# Autodesk Inventor assembly: Backhoe
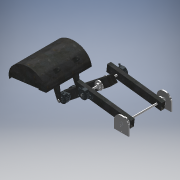
[picture p0: Inventor's stored thumbnail of the model, 180x180]
Saved by Autodesk Inventor 2019 (Build 230136000, 136)
## iProperties
Created: 2018-10-28
Part Number: Backhoe
Document SubType Name: Assembly
Designer: Alex Barnett
Author: Alex Barnett
## Documents named in this file (11)
- C:\Users\Alex Barnett\Documents\Machine Design\PR2\CAD\Backhoe.iam
- C:\Users\Alex Barnett\Documents\Machine Design\PR2\CAD\Boom Hinge.ipt
- C:\Users\Alex Barnett\Documents\Machine Design\PR2\CAD\Pin .5in. Dia. - Boom Hinge.ipt
- C:\Users\Alex Barnett\Documents\Machine Design\PR2\CAD\Ball Bearing .5in..ipt
- C:\Users\Alex Barnett\Documents\Machine Design\PR2\CAD\Steel 4130 1x2in. Tubing, t=.065in.,L=15in..ipt
- C:\Users\Alex Barnett\Documents\Machine Design\PR2\CAD\Flange-Mount Shaft Collar 0.5in..ipt
- C:\Users\Alex Barnett\Documents\Machine Design\PR2\CAD\Steel 4130 1x2in. Tubing, t=.065in.,L=22in..ipt
- C:\Users\Alex Barnett\Documents\Machine Design\PR2\CAD\Flange-Mount Sealed Ball Bearing .5in. Dia..ipt
- C:\Users\Alex Barnett\Documents\Machine Design\PR2\CAD\Boom to Stick .5in. Pin.ipt
- C:\Users\Alex Barnett\Documents\Machine Design\PR2\CAD\Stick to Scoop .5in. Pin.ipt
- C:\Users\Alex Barnett\Documents\Machine Design\PR2\CAD\Bucket.ipt
## Components (20 placed, 10 different names)
1. Boom Hinge:1 — Mate:1, Mate:2, Mate:3, Flush:2, Mate:6, Mate:7, Flush:3, Mate:14, Mate:26
2. Boom Hinge:2 — Mate:5, Flush:2, Mate:8, Flush:4, Flush:5, Mate:14, Mate:19, Mate:54, Flush:11
3. Pin .5in. Dia. - Boom Hinge:1 — Mate:5, Mate:6, Flush:5, Mate:15, Mate:21, Mate:22, Mate:54
4. Ball Bearing .5in.:1 — Mate:7, Flush:3
5. Ball Bearing .5in.:2 — Mate:8, Flush:4
6. Steel 4130 1x2in. Tubing, t=.065in.,L=15in.:1 — Flush:6, Mate:21, Mate:23, Mate:24, Mate:27, Mate:32, Mate:33, Mate:34
7. Flange-Mount Shaft Collar 0.5in.:2 — Mate:15, Mate:16, Mate:17, Mate:18, Mate:19
8. Steel 4130 1x2in. Tubing, t=.065in.,L=15in.:2 — Mate:16, Mate:17, Mate:18, Flush:6, Mate:20, Mate:29, Mate:30, Mate:31, Flush:9
9. Steel 4130 1x2in. Tubing, t=.065in.,L=22in.:1 — Mate:20, Flush:7, Mate:38, Mate:39, Mate:40, Mate:41, Flush:9, Mate:46, Mate:47, Mate:48, Flush:10
10. Flange-Mount Shaft Collar 0.5in.:3 — Mate:22, Mate:23, Mate:24, Mate:26
11. Steel 4130 1x2in. Tubing, t=.065in.,L=22in.:2 — Mate:27, Flush:7, Mate:41, Mate:43, Mate:44, Mate:45, Mate:49, Mate:50, Mate:51
12. Flange-Mount Sealed Ball Bearing .5in. Dia.:1 — Mate:29, Mate:30, Mate:31, Mate:35, Flush:8
13. Flange-Mount Sealed Ball Bearing .5in. Dia.:2 — Mate:32, Mate:33, Mate:34
14. Boom to Stick .5in. Pin:1 — Mate:35, Flush:8, Mate:36, Mate:42
15. Flange-Mount Shaft Collar 0.5in.:4 — Mate:36, Mate:38, Mate:39, Mate:40
16. Flange-Mount Shaft Collar 0.5in.:5 — Mate:42, Mate:43, Mate:44, Mate:45
17. Flange-Mount Sealed Ball Bearing .5in. Dia.:3 — Mate:46, Mate:47, Mate:48, Mate:52
18. Flange-Mount Sealed Ball Bearing .5in. Dia.:4 — Mate:49, Mate:50, Mate:51, Mate:61
19. Stick to Scoop .5in. Pin:1 — Mate:52, Flush:10, Mate:60
20. Bucket:1 — Mate:60, Mate:61
## Relationships (58: Mate 46, Flush 12)
- Mate:1: Boom Hinge:1
- Mate:2: Boom Hinge:1
- Mate:3: Boom Hinge:1
- Mate:5: Boom Hinge:2 ↔ Pin .5in. Dia. - Boom Hinge:1
- Flush:2: Boom Hinge:1 ↔ Boom Hinge:2
- Mate:6: Boom Hinge:1 ↔ Pin .5in. Dia. - Boom Hinge:1
- Mate:7: Boom Hinge:1 ↔ Ball Bearing .5in.:1
- Flush:3: Boom Hinge:1 ↔ Ball Bearing .5in.:1
- Mate:8: Boom Hinge:2 ↔ Ball Bearing .5in.:2
- Flush:4: Boom Hinge:2 ↔ Ball Bearing .5in.:2
- Flush:5: Boom Hinge:2 ↔ Pin .5in. Dia. - Boom Hinge:1
- Mate:14 (-304.8 mm): Boom Hinge:1 ↔ Boom Hinge:2
- Mate:15: Pin .5in. Dia. - Boom Hinge:1 ↔ Flange-Mount Shaft Collar 0.5in.:2
- Mate:16: Flange-Mount Shaft Collar 0.5in.:2 ↔ Steel 4130 1x2in. Tubing, t=.065in.,L=15in.:2
- Mate:17: Flange-Mount Shaft Collar 0.5in.:2 ↔ Steel 4130 1x2in. Tubing, t=.065in.,L=15in.:2
- Mate:18: Flange-Mount Shaft Collar 0.5in.:2 ↔ Steel 4130 1x2in. Tubing, t=.065in.,L=15in.:2
- Flush:6: Steel 4130 1x2in. Tubing, t=.065in.,L=15in.:1 ↔ Steel 4130 1x2in. Tubing, t=.065in.,L=15in.:2
- Mate:19 (6.35 mm): Boom Hinge:2 ↔ Flange-Mount Shaft Collar 0.5in.:2
- Mate:20: Steel 4130 1x2in. Tubing, t=.065in.,L=15in.:2 ↔ Steel 4130 1x2in. Tubing, t=.065in.,L=22in.:1
- Mate:21: Pin .5in. Dia. - Boom Hinge:1 ↔ Steel 4130 1x2in. Tubing, t=.065in.,L=15in.:1
- Mate:22: Pin .5in. Dia. - Boom Hinge:1 ↔ Flange-Mount Shaft Collar 0.5in.:3
- Mate:23: Steel 4130 1x2in. Tubing, t=.065in.,L=15in.:1 ↔ Flange-Mount Shaft Collar 0.5in.:3
- Mate:24: Steel 4130 1x2in. Tubing, t=.065in.,L=15in.:1 ↔ Flange-Mount Shaft Collar 0.5in.:3
- Mate:26 (6.35 mm): Boom Hinge:1 ↔ Flange-Mount Shaft Collar 0.5in.:3
- Mate:27: Steel 4130 1x2in. Tubing, t=.065in.,L=15in.:1 ↔ Steel 4130 1x2in. Tubing, t=.065in.,L=22in.:2
- Flush:7: Steel 4130 1x2in. Tubing, t=.065in.,L=22in.:1 ↔ Steel 4130 1x2in. Tubing, t=.065in.,L=22in.:2
- Mate:29: Steel 4130 1x2in. Tubing, t=.065in.,L=15in.:2 ↔ Flange-Mount Sealed Ball Bearing .5in. Dia.:1
- Mate:30: Steel 4130 1x2in. Tubing, t=.065in.,L=15in.:2 ↔ Flange-Mount Sealed Ball Bearing .5in. Dia.:1
- Mate:31: Steel 4130 1x2in. Tubing, t=.065in.,L=15in.:2 ↔ Flange-Mount Sealed Ball Bearing .5in. Dia.:1
- Mate:32: Steel 4130 1x2in. Tubing, t=.065in.,L=15in.:1 ↔ Flange-Mount Sealed Ball Bearing .5in. Dia.:2
- Mate:33: Steel 4130 1x2in. Tubing, t=.065in.,L=15in.:1 ↔ Flange-Mount Sealed Ball Bearing .5in. Dia.:2
- Mate:34: Steel 4130 1x2in. Tubing, t=.065in.,L=15in.:1 ↔ Flange-Mount Sealed Ball Bearing .5in. Dia.:2
- Mate:35: Flange-Mount Sealed Ball Bearing .5in. Dia.:1 ↔ Boom to Stick .5in. Pin:1
- Flush:8: Flange-Mount Sealed Ball Bearing .5in. Dia.:1 ↔ Boom to Stick .5in. Pin:1
- Mate:36: Boom to Stick .5in. Pin:1 ↔ Flange-Mount Shaft Collar 0.5in.:4
- Mate:38: Steel 4130 1x2in. Tubing, t=.065in.,L=22in.:1 ↔ Flange-Mount Shaft Collar 0.5in.:4
- Mate:39: Steel 4130 1x2in. Tubing, t=.065in.,L=22in.:1 ↔ Flange-Mount Shaft Collar 0.5in.:4
- Mate:40: Steel 4130 1x2in. Tubing, t=.065in.,L=22in.:1 ↔ Flange-Mount Shaft Collar 0.5in.:4
- Mate:41: Steel 4130 1x2in. Tubing, t=.065in.,L=22in.:1 ↔ Steel 4130 1x2in. Tubing, t=.065in.,L=22in.:2
- Mate:42: Boom to Stick .5in. Pin:1 ↔ Flange-Mount Shaft Collar 0.5in.:5
- Mate:43: Steel 4130 1x2in. Tubing, t=.065in.,L=22in.:2 ↔ Flange-Mount Shaft Collar 0.5in.:5
- Mate:44: Steel 4130 1x2in. Tubing, t=.065in.,L=22in.:2 ↔ Flange-Mount Shaft Collar 0.5in.:5
- Mate:45: Steel 4130 1x2in. Tubing, t=.065in.,L=22in.:2 ↔ Flange-Mount Shaft Collar 0.5in.:5
- Flush:9 (119.0625 mm): Steel 4130 1x2in. Tubing, t=.065in.,L=15in.:2 ↔ Steel 4130 1x2in. Tubing, t=.065in.,L=22in.:1
- Mate:46: Steel 4130 1x2in. Tubing, t=.065in.,L=22in.:1 ↔ Flange-Mount Sealed Ball Bearing .5in. Dia.:3
- Mate:47: Steel 4130 1x2in. Tubing, t=.065in.,L=22in.:1 ↔ Flange-Mount Sealed Ball Bearing .5in. Dia.:3
- Mate:48: Steel 4130 1x2in. Tubing, t=.065in.,L=22in.:1 ↔ Flange-Mount Sealed Ball Bearing .5in. Dia.:3
- Mate:49: Steel 4130 1x2in. Tubing, t=.065in.,L=22in.:2 ↔ Flange-Mount Sealed Ball Bearing .5in. Dia.:4
- Mate:50: Steel 4130 1x2in. Tubing, t=.065in.,L=22in.:2 ↔ Flange-Mount Sealed Ball Bearing .5in. Dia.:4
- Mate:51: Steel 4130 1x2in. Tubing, t=.065in.,L=22in.:2 ↔ Flange-Mount Sealed Ball Bearing .5in. Dia.:4
- Mate:52: Flange-Mount Sealed Ball Bearing .5in. Dia.:3 ↔ Stick to Scoop .5in. Pin:1
- Flush:10: Steel 4130 1x2in. Tubing, t=.065in.,L=22in.:1 ↔ Stick to Scoop .5in. Pin:1
- Mate:54: Boom Hinge:2 ↔ Pin .5in. Dia. - Boom Hinge:1
- Flush:11: Boom Hinge:2
- Flush:12 (300 mm)
- Flush:13 (500 mm)
- Mate:60: Stick to Scoop .5in. Pin:1 ↔ Bucket:1
- Mate:61 (6.35 mm): Flange-Mount Sealed Ball Bearing .5in. Dia.:4 ↔ Bucket:1
